# Autodesk Inventor assembly: Assembly
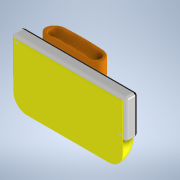
[picture p0: Inventor's stored thumbnail of the model, 180x180]
Saved by Autodesk Inventor 2021 (Build 250183000, 183)
## iProperties
Created: 2021-03-30
Part Number: Assembly
Document SubType Name: Assembly
Designer: eng1-177
Author: eng1-177
## Documents named in this file (7)
- C:\Users\eng1-177\Desktop\Refined Design\Assembly.iam
- C:\Users\eng1-177\Desktop\Base.ipt
- C:\Users\eng1-177\Desktop\Handle.ipt
- C:\Users\eng1-177\Desktop\Cover.ipt
- C:\Users\eng1-177\Desktop\Wrist Rest.ipt
- C:\Users\eng1-177\Desktop\UP Button.ipt
- C:\Users\eng1-177\Desktop\DOWN Button.ipt
## Components (6 placed, 6 different names)
1. Base:1 — Mate:1, Ball:1, Mate:2, Mate:3, Mate:4, Insert:1, Insert:2
2. Handle:1 — Mate:1, Ball:1
3. Cover:1 — Mate:2, Mate:3, Mate:4, Mate:5, Mate:6, Mate:7
4. Wrist Rest:1 — Insert:1
5. UP Button:1 — Mate:5, Mate:6
6. DOWN Button:1 — Mate:7, Insert:2
## Relationships (10: Mate 7, Insert 2, BallJoint 1)
- Mate:1: Base:1 ↔ Handle:1
- Ball:1: Base:1 ↔ Handle:1
- Mate:2: Base:1 ↔ Cover:1
- Mate:3: Base:1 ↔ Cover:1
- Mate:4: Base:1 ↔ Cover:1
- Insert:1: Base:1 ↔ Wrist Rest:1
- Mate:5: Cover:1 ↔ UP Button:1
- Mate:6: Cover:1 ↔ UP Button:1
- Mate:7: Cover:1 ↔ DOWN Button:1
- Insert:2: Base:1 ↔ DOWN Button:1
